# Autodesk Inventor assembly: Vex Arm, Second Draft
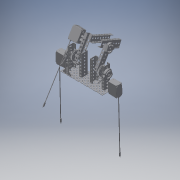
[picture p0: Inventor's stored thumbnail of the model, 180x180]
Saved by Autodesk Inventor 2018 (Build 220112000, 112)
## iProperties
Created: 2017-06-28
Part Number: Vex Arm, Second Draft
Document SubType Name: Assembly
Designer: James
Author: James
## Documents named in this file (10)
- C:\Users\James\Desktop\EE REU\Hardware\Vex Arm\Vex Arm Draft 2\Vex Arm, climbing edition.iam
- C:\Users\James\Desktop\EE REU\Hardware\Vex Arm\Vex Arm Draft 2\Base (Draft 2).iam
- C:\Users\James\Desktop\EE REU\Hardware\Vex Arm\Vex Arm Draft 2\First Base Extension (Draft 2).iam
- C:\Users\James\Desktop\EE REU\Hardware\Vex Arm\Vex Arm Draft 2\Second Base Extension (Draft 2).iam
- C:\Users\James\Desktop\EE REU\Hardware\Vex Arm\Vex Parts\MOTION-MODEL-PACK\SHAFT-COLLAR.ipt
- C:\Users\James\Desktop\EE REU\Hardware\Vex Arm\Vex Parts\Vex Potentiometer.ipt
- C:\Users\James\Desktop\EE REU\Hardware\Vex Arm\Vex Parts\Vex Hardware and Metal Kit\BEARING-FLAT.ipt
- C:\Users\James\Desktop\EE REU\Hardware\Vex Arm\Vex Parts\Vex Hardware and Metal Kit\VL-PLATE-5-15 RevA.ipt
- C:\Users\James\Desktop\EE REU\Hardware\Vex Arm\Vex Parts\Base C Channel.ipt
- C:\Users\James\Desktop\EE REU\Hardware\Vex Arm\Vex Parts\Vex Hardware and Metal Kit\ANGLE-GUSSET.ipt
## Components (13 placed, 9 different names)
1. Base (Draft 2):1 [sub-assembly] — Insert:1, Insert:9, Insert:10, Mate:1, Flush:1, Flush:2, Mate:2, Flush:3, Flush:4, Mate:3, Flush:5, Insert:11
2. First Base Extension (Draft 2):1 [sub-assembly] — Insert:1, Insert:2, Insert:3, Insert:4, Insert:5
3. Second Base Extension (Draft 2):1 [sub-assembly] — Insert:5
4. SHAFT-COLLAR:1 — Insert:3
5. SHAFT-COLLAR:2 — Insert:2
6. Vex Potentiometer:1 — Insert:4
7. BEARING-FLAT:1 — Insert:9
8. BEARING-FLAT:2 — Insert:10
9. VL-PLATE-5-15 RevA:1 — Mate:1, Flush:1, Mate:4
10. Base C Channel:1 — Flush:2, Mate:2, Flush:3
11. Base C Channel:2 — Flush:4, Mate:3, Flush:5
12. Vex Potentiometer:2 — Insert:11
13. ANGLE-GUSSET:3 — Mate:4
## Relationships (17: Insert 8, Flush 5, Mate 4)
- Insert:1: Base (Draft 2):1 ↔ First Base Extension (Draft 2):1
- Insert:2: First Base Extension (Draft 2):1 ↔ SHAFT-COLLAR:2
- Insert:3: First Base Extension (Draft 2):1 ↔ SHAFT-COLLAR:1
- Insert:4: First Base Extension (Draft 2):1 ↔ Vex Potentiometer:1
- Insert:5 (25 mm): First Base Extension (Draft 2):1 ↔ Second Base Extension (Draft 2):1
- Insert:9: Base (Draft 2):1 ↔ BEARING-FLAT:1
- Insert:10: Base (Draft 2):1 ↔ BEARING-FLAT:2
- Mate:1 (-50 mm): Base (Draft 2):1 ↔ VL-PLATE-5-15 RevA:1
- Flush:1 (-10 mm): Base (Draft 2):1 ↔ VL-PLATE-5-15 RevA:1
- Flush:2: Base (Draft 2):1 ↔ Base C Channel:1
- Mate:2 (60 mm): Base (Draft 2):1 ↔ Base C Channel:1
- Flush:3: Base (Draft 2):1 ↔ Base C Channel:1
- Flush:4: Base (Draft 2):1 ↔ Base C Channel:2
- Mate:3 (60 mm): Base (Draft 2):1 ↔ Base C Channel:2
- Flush:5: Base (Draft 2):1 ↔ Base C Channel:2
- Insert:11: Base (Draft 2):1 ↔ Vex Potentiometer:2
- Mate:4: VL-PLATE-5-15 RevA:1 ↔ ANGLE-GUSSET:3
